# Autodesk Inventor assembly: Assembly1
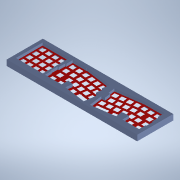
[picture p0: Inventor's stored thumbnail of the model, 180x180]
Saved by Autodesk Inventor 2020 (Build 240168000, 168)
## iProperties
Created: 2019-06-10
Part Number: Assembly1
Document SubType Name: Assembly
Designer: Holt
Author: Holt
## Documents named in this file (4)
- C:\Users\Holt\OneDrive\Keyboard Stuff\BLE_Feather\Adafruit Feather 32u4 Bluefruit LE\CAD\Assembly1.iam
- C:\Users\Holt\OneDrive\Keyboard Stuff\BLE_Feather\Adafruit Feather 32u4 Bluefruit LE\CAD\Prime_BLE_Top.ipt
- C:\Users\Holt\OneDrive\Keyboard Stuff\BLE_Feather\Adafruit Feather 32u4 Bluefruit LE\CAD\switch plate.ipt
- C:\Users\Holt\OneDrive\Keyboard Stuff\BLE_Feather\Adafruit Feather 32u4 Bluefruit LE\CAD\bottom.ipt
## Components (3 placed, 3 different names)
1. Prime_BLE_Top:1 — Mate:1, Mate:2, Mate:3, Mate:8, Flush:1, Flush:2
2. switch plate:1 — Mate:1, Mate:2, Mate:3
3. bottom:1 — Mate:8, Flush:1, Flush:2
## Relationships (6: Mate 4, Flush 2)
- Mate:1: Prime_BLE_Top:1 ↔ switch plate:1
- Mate:2: Prime_BLE_Top:1 ↔ switch plate:1
- Mate:3: Prime_BLE_Top:1 ↔ switch plate:1
- Mate:8: Prime_BLE_Top:1 ↔ bottom:1
- Flush:1: Prime_BLE_Top:1 ↔ bottom:1
- Flush:2: Prime_BLE_Top:1 ↔ bottom:1
